# Autodesk Inventor assembly: AssyCage
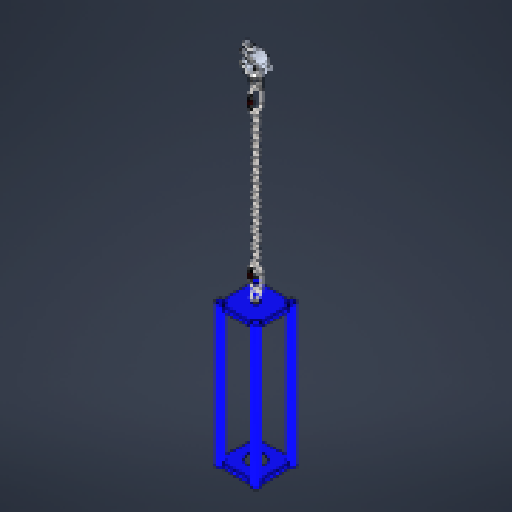
[picture p0: Inventor's stored thumbnail of the model, 512x512]
Saved by Autodesk Inventor 2024.3 (Build 283343000, 343)
## iProperties
Created: 2025-03-16
Part Number: AssyCage
Document SubType Name: Assembly
Designer: jings
Author: jings
## Documents named in this file (3)
- C:\Users\jings\OneDrive\Desktop\2025-Poseidon-Mechanical\5_Field\Cage\AssyCage.iam
- C:\Users\jings\Downloads\CageChainOnly\CageChainOnly\CageChainOnly.ipt
- C:\Users\jings\Downloads\CageNoChain\CageNoChain\CageNoChain.ipt
## Components (2 placed, 2 different names)
1. CageChainOnly:1 — Ball:1
2. CageNoChain:1 — Ball:1
## Relationships (1: BallJoint 1)
- Ball:1: CageChainOnly:1 ↔ CageNoChain:1
